# Autodesk Inventor assembly: ASM_Micron_All_Assembled
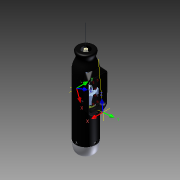
[picture p0: Inventor's stored thumbnail of the model, 180x180]
Saved by Autodesk Inventor 2011 SP2 (Build 150309200, 309)
## iProperties
Created: 2011-10-07
Part Number: ASM_Micron_All_Assembled
Document SubType Name: Assembly
Designer: sungwook
Author: sungwook
## Documents named in this file (13)
- C:\Users\sungwook\Documents\Inventor\Micron22_top_adj_02082013\06242013_FigGen\ASM_Micron_All_Assembled.iam
- C:\Users\sungwook\Documents\Inventor\Micron22_top_adj_02082013\Assembly\Motion_Merge\Indep\ASM_Micron_ASAP_Indep0.iam
- C:\Users\sungwook\Documents\Inventor\Micron22_top_adj_02082013\Parts\ASAP\Handle_ASAP.iam
- C:\Users\sungwook\Documents\Inventor\Micron22_top_adj_02082013\Parts\Electronics\PCB_Stack.iam
- C:\Users\sungwook\Documents\Inventor\Micron22_top_adj_02082013\06082012_Outer_Tube\Outer_Tube.ipt
- C:\Users\sungwook\Documents\Inventor\Content Center Files\R2011\en-US\ANSI B18.6.3(00)\ANSI B18.6.3 - 0-80 UNF - 0.1875(32).ipt
- C:\Users\sungwook\Documents\Inventor\Micron22_top_adj_02082013\Parts\Handle\Ver2(Al_RP)\Handle_2_Back_rev2.ipt
- C:\Users\sungwook\Documents\Inventor\Micron22_top_adj_02082013\04192012_New_Front_2pcs\New_Front_Base_rev.ipt
- C:\Users\sungwook\Documents\Inventor\Micron22_top_adj_02082013\04192012_New_Front_2pcs\New_Front_Upper_rev_v2.ipt
- C:\Users\sungwook\Documents\Inventor\Micron22_top_adj_02082013\Parts\Tool\Needle_Asm.iam
- C:\Users\sungwook\Documents\Inventor\Micron22_top_adj_02082013\Parts\Tool\Tool Mount_Rev.ipt
- C:\Users\sungwook\Documents\Inventor\Micron22_top_adj_02082013\Parts\Tool\Tool_Mount_Luer_Adapter.ipt
- C:\Users\sungwook\Documents\Inventor\Micron22_top_adj_02082013\Parts\Handle\Guide_Tubing.ipt
## Components (14 placed, 12 different names)
1. (0,0,0) [sub-assembly] — Mate:2, Mate:55, Mate:73, Mate:74, Mate:107, Mate:108, Mate:125, Mate:126, Mate:127, Mate:128, Mate:130
2. Handle_ASAP:1 [sub-assembly] — Mate:55
3. PCB_Stack:1 [sub-assembly] — Flush:73, Mate:73, Mate:74
4. Needle_Asm:1 [sub-assembly] — Mate:124, Mate:132
5. Tool Mount_Rev:1 — Mate:122, Mate:123, Mate:126, Mate:127, Mate:128, Mate:132
6. Tool_Mount_Luer_Adapter:1 — Mate:122, Mate:123, Mate:124, Mate:125
7. Guide_Tubing:1 — Mate:129, Flush:123
8. New_Front_Base_rev:1 — Mate:112, Mate:113, Mate:114, Mate:120, Flush:121
9. New_Front_Upper_rev_v2:1 — Mate:120, Flush:121, Flush:122
10. Handle_2_Back_rev2:1 — Mate:109, Mate:110, Mate:111, Mate:129, Flush:123, Mate:131
11. Outer_Tube:1 — Mate:104, Mate:105, Mate:108, Mate:109, Mate:111, Mate:114, Flush:122, Mate:130, Mate:131
12. Cross Recessed 100° Flat Countersunk Head Machine Screw - Type I - Inch 0-80 UNF x 0.1875:1 — Mate:107
13. Cross Recessed 100° Flat Countersunk Head Machine Screw - Type I - Inch 0-80 UNF x 0.1875:2
14. Cross Recessed 100° Flat Countersunk Head Machine Screw - Type I - Inch 0-80 UNF x 0.1875:3
## Component patterns: (3 elements, first: Cross Recessed 100° Flat Countersunk Head Machine Screw - Type I - Inch 0-80 UNF x 0.1875:1)
## Relationships (30: Mate 26, Flush 4)
- Mate:2: (0,0,0)
- Mate:55: (0,0,0) ↔ Handle_ASAP:1
- Flush:73: PCB_Stack:1
- Mate:73: (0,0,0) ↔ PCB_Stack:1
- Mate:74: (0,0,0) ↔ PCB_Stack:1
- Mate:104: Outer_Tube:1
- Mate:105: Outer_Tube:1
- Mate:108: (0,0,0) ↔ Outer_Tube:1
- Mate:109: Handle_2_Back_rev2:1 ↔ Outer_Tube:1
- Mate:110: Handle_2_Back_rev2:1
- Mate:111: Handle_2_Back_rev2:1 ↔ Outer_Tube:1
- Mate:112: New_Front_Base_rev:1
- Mate:113: New_Front_Base_rev:1
- Mate:114: New_Front_Base_rev:1 ↔ Outer_Tube:1
- Mate:120: New_Front_Base_rev:1 ↔ New_Front_Upper_rev_v2:1
- Flush:121: New_Front_Base_rev:1 ↔ New_Front_Upper_rev_v2:1
- Flush:122: New_Front_Upper_rev_v2:1 ↔ Outer_Tube:1
- Mate:122: Tool Mount_Rev:1 ↔ Tool_Mount_Luer_Adapter:1
- Mate:123: Tool Mount_Rev:1 ↔ Tool_Mount_Luer_Adapter:1
- Mate:124: Needle_Asm:1 ↔ Tool_Mount_Luer_Adapter:1
- Mate:125: (0,0,0) ↔ Tool_Mount_Luer_Adapter:1
- Mate:126: (0,0,0) ↔ Tool Mount_Rev:1
- Mate:127: (0,0,0) ↔ Tool Mount_Rev:1
- Mate:128: (0,0,0) ↔ Tool Mount_Rev:1
- Mate:129: Guide_Tubing:1 ↔ Handle_2_Back_rev2:1
- Mate:130: (0,0,0) ↔ Outer_Tube:1
- Flush:123 (2 mm): Guide_Tubing:1 ↔ Handle_2_Back_rev2:1
- Mate:131: Handle_2_Back_rev2:1 ↔ Outer_Tube:1
- Mate:132 (3 mm): Needle_Asm:1 ↔ Tool Mount_Rev:1
- Mate:107: (0,0,0) ↔ Cross Recessed 100° Flat Countersunk Head Machine Screw - Type I - Inch 0-80 UNF x 0.1875:1
